# Autodesk Inventor assembly: Middle Pulley Assembly
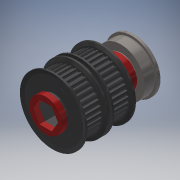
[picture p0: Inventor's stored thumbnail of the model, 180x180]
Saved by Autodesk Inventor 2018 (Build 220112000, 112)
## iProperties
Created: 2018-12-20
Part Number: Middle Pulley Assembly
Document SubType Name: Assembly
Designer: maste
Author: maste
## Documents named in this file (4)
- F:\Summer Drive Base V1\Summer Drivebase\Middle Pulley Assembly.iam
- F:\Summer Drive Base V1\Summer Drivebase\36t_x_9mm_Wide_Double_Flange_Aluminum_Pulley_GT2_3mm_1_2_Hex_Bore_217-5873.ipt
- F:\Summer Drive Base V1\Summer Drivebase\0.125in Spacer.ipt
- F:\Summer Drive Base V1\Summer Drivebase\0_500_Hex_ID_x_1_125_OD_x_0_313_WD_Flanged_Bearing_v2_217-3875.ipt
## Components (7 placed, 3 different names)
1. 36t_x_9mm_Wide_Double_Flange_Aluminum_Pulley_GT2_3mm_1_2_Hex_Bore_217-5873:3 — Mate:1, Flush:1, Flush:2, Mate:2, Flush:3, Flush:4
2. 36t_x_9mm_Wide_Double_Flange_Aluminum_Pulley_GT2_3mm_1_2_Hex_Bore_217-5873:4 — Mate:2, Flush:3, Flush:4, Mate:3, Flush:5, Flush:6
3. 0.125in Spacer:5 — Mate:1, Flush:1, Flush:2
4. 0.125in Spacer:6 — Mate:3, Flush:5, Flush:6, Mate:4, Flush:7, Flush:8
5. 0.125in Spacer:7 — Mate:4, Flush:7, Flush:8, Mate:5, Flush:9, Flush:10
6. 0.125in Spacer:8 — Mate:5, Flush:9, Flush:10, Mate:6, Flush:11, Flush:12
7. 0_500_Hex_ID_x_1_125_OD_x_0_313_WD_Flanged_Bearing_v2_217-3875:1 — Mate:6, Flush:11, Flush:12
## Relationships (18: Flush 12, Mate 6)
- Mate:1: 36t_x_9mm_Wide_Double_Flange_Aluminum_Pulley_GT2_3mm_1_2_Hex_Bore_217-5873:3 ↔ 0.125in Spacer:5
- Flush:1: 36t_x_9mm_Wide_Double_Flange_Aluminum_Pulley_GT2_3mm_1_2_Hex_Bore_217-5873:3 ↔ 0.125in Spacer:5
- Flush:2: 36t_x_9mm_Wide_Double_Flange_Aluminum_Pulley_GT2_3mm_1_2_Hex_Bore_217-5873:3 ↔ 0.125in Spacer:5
- Mate:2: 36t_x_9mm_Wide_Double_Flange_Aluminum_Pulley_GT2_3mm_1_2_Hex_Bore_217-5873:3 ↔ 36t_x_9mm_Wide_Double_Flange_Aluminum_Pulley_GT2_3mm_1_2_Hex_Bore_217-5873:4
- Flush:3: 36t_x_9mm_Wide_Double_Flange_Aluminum_Pulley_GT2_3mm_1_2_Hex_Bore_217-5873:3 ↔ 36t_x_9mm_Wide_Double_Flange_Aluminum_Pulley_GT2_3mm_1_2_Hex_Bore_217-5873:4
- Flush:4: 36t_x_9mm_Wide_Double_Flange_Aluminum_Pulley_GT2_3mm_1_2_Hex_Bore_217-5873:3 ↔ 36t_x_9mm_Wide_Double_Flange_Aluminum_Pulley_GT2_3mm_1_2_Hex_Bore_217-5873:4
- Mate:3: 36t_x_9mm_Wide_Double_Flange_Aluminum_Pulley_GT2_3mm_1_2_Hex_Bore_217-5873:4 ↔ 0.125in Spacer:6
- Flush:5: 36t_x_9mm_Wide_Double_Flange_Aluminum_Pulley_GT2_3mm_1_2_Hex_Bore_217-5873:4 ↔ 0.125in Spacer:6
- Flush:6: 36t_x_9mm_Wide_Double_Flange_Aluminum_Pulley_GT2_3mm_1_2_Hex_Bore_217-5873:4 ↔ 0.125in Spacer:6
- Mate:4: 0.125in Spacer:6 ↔ 0.125in Spacer:7
- Flush:7: 0.125in Spacer:6 ↔ 0.125in Spacer:7
- Flush:8: 0.125in Spacer:6 ↔ 0.125in Spacer:7
- Mate:5: 0.125in Spacer:7 ↔ 0.125in Spacer:8
- Flush:9: 0.125in Spacer:7 ↔ 0.125in Spacer:8
- Flush:10: 0.125in Spacer:7 ↔ 0.125in Spacer:8
- Mate:6: 0.125in Spacer:8 ↔ 0_500_Hex_ID_x_1_125_OD_x_0_313_WD_Flanged_Bearing_v2_217-3875:1
- Flush:11: 0.125in Spacer:8 ↔ 0_500_Hex_ID_x_1_125_OD_x_0_313_WD_Flanged_Bearing_v2_217-3875:1
- Flush:12: 0.125in Spacer:8 ↔ 0_500_Hex_ID_x_1_125_OD_x_0_313_WD_Flanged_Bearing_v2_217-3875:1
